# Autodesk Inventor assembly: Assembly4
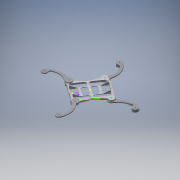
[picture p0: Inventor's stored thumbnail of the model, 180x180]
Saved by Autodesk Inventor 2016 (Build 200138000, 138)
## iProperties
Created: 2016-01-12
Part Number: Assembly4
Document SubType Name: Assembly
Designer: cemer
Author: cemer
## Documents named in this file (6)
- C:\Users\cemer\Desktop\Assembly4.iam
- C:\Users\cemer\Desktop\Part4.ipt
- C:\Users\cemer\Desktop\Part3.ipt
- C:\Users\cemer\Desktop\Part1.ipt
- C:\Users\cemer\Desktop\Part4_MIR.ipt
- C:\Users\cemer\Desktop\Part3_MIR.ipt
## Components (5 placed, 5 different names)
1. Part4:2 — Rotational:1
2. Part3:2 — Rotational:5
3. Part1:1 — Rotational:1, Rotational:3, Rotational:4, Rotational:5
4. Part4_MIR:1 — Rotational:3
5. Part3_MIR:1 — Rotational:4
## Relationships (4: RevoluteJoint 4)
- Rotational:1 [RevoluteJoint]: Part4:2 ↔ Part1:1
- Rotational:3 [RevoluteJoint]: Part1:1 ↔ Part4_MIR:1
- Rotational:4 [RevoluteJoint]: Part1:1 ↔ Part3_MIR:1
- Rotational:5 [RevoluteJoint]: Part3:2 ↔ Part1:1
